# Autodesk Inventor assembly: ASS - 2021 - CUBLEND40F50 - V04
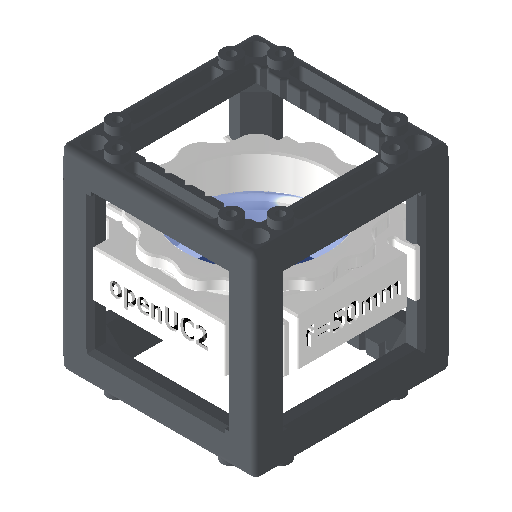
[picture p0: Inventor's stored thumbnail of the model, 512x512]
Saved by Autodesk Inventor 2025.1 (Build 291241000, 241)
## iProperties
Created: 2025-01-02
Part Number: ASS - 2021 - CUBLEND40F50 - V04
Document SubType Name: Assembly
Designer: Gerstenberger
Description: Cube with lens f = 50 mm
Mass: 52.4266 g
Surface Area: 330.33 cm^2
Volume: 43.9542 cm^3
Density: 1.19276 g/cm^3
Author: Gerstenberger
## Documents named in this file (3)
- C:\UC2\openUC2-CAD-new\Workspace\ASS\ASS - 2021 - CUBLEND40F50 - V04.iam
- C:\UC2\openUC2-CAD-new\Workspace\PRT\PRT - 1003 - CUBHLF111 - V04.ipt
- C:\UC2\openUC2-CAD-new\Workspace\SUB\SUB - 0023 - LEND40F50 - V04 - virt ass.iam
## Components (3 placed, 2 different names)
1. SUB - 0023 - LEND40F50 - V04 - virt ass:1 [sub-assembly] — Passend:1, Winkel:1, Winkel:2, Winkel:3, Winkel:4
2. PRT - 1003 - CUBHLF111 - V04:1
3. PRT - 1003 - CUBHLF111 - V04:2
## Component patterns: (2 elements, first: PRT - 1003 - CUBHLF111 - V04:1)
## Relationships (5: Angle 4, Mate 1)
- Passend:1 [Mate]: SUB - 0023 - LEND40F50 - V04 - virt ass:1
- Winkel:1 [Angle] (0 deg): SUB - 0023 - LEND40F50 - V04 - virt ass:1
- Winkel:2 [Angle] (0 deg): SUB - 0023 - LEND40F50 - V04 - virt ass:1
- Winkel:3 [Angle] (180 deg): SUB - 0023 - LEND40F50 - V04 - virt ass:1
- Winkel:4 [Angle] (0 deg): SUB - 0023 - LEND40F50 - V04 - virt ass:1
